# Autodesk Inventor assembly: GE-12053
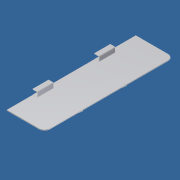
[picture p0: Inventor's stored thumbnail of the model, 180x180]
Saved by Autodesk Inventor 2012 (Build 160160000, 160)
## iProperties
Created: 2011-08-29
Part Number: GE-12053
Document SubType Name: Assembly
Designer: mcyr
Description: Shelf Assembly
Title: Shelf Assembly
Author: mcyr
## Documents named in this file (5)
- C:\Data Folder\FRC 2012 Field\Components\GE-12053.iam
- C:\Data Folder\FRC 2012 Field\Components\GE-12053-02.ipt
- C:\Data Folder\FRC 2012 Field\Components\GE-12053-01.ipt
- C:\Data Folder\FRC 2012 Field\Components\FE-00004-08.iam
- C:\Data Folder\FRC 2012 Field\Components\GE-12052_modified.ipt
## Components (7 placed, 4 different names)
1. GE-12053-02:1 — Mate:1, Flush:1, Mate:2, Flush:2, Flush:3, Mate:4, Flush:4
2. GE-12053-02:2 — Mate:2, Mate:3, Flush:3, Mate:7, Flush:5
3. GE-12053-01:1 — Mate:1, Flush:1, Mate:3, Flush:2, Mate:5, Mate:6, Flush:8, Flush:9, Mate:9, Flush:10, Mate:10, Flush:11
4. FE-00004-08:1 [sub-assembly] — Mate:6, Mate:7, Flush:5
5. FE-00004-08:2 [sub-assembly] — Mate:4, Mate:5, Flush:4
6. GE-12052_modified:1 — Flush:9, Mate:10, Flush:11
7. GE-12052_modified:2 — Flush:8, Mate:9, Flush:10
## Relationships (18: Mate 9, Flush 9)
- Mate:1: GE-12053-02:1 ↔ GE-12053-01:1
- Flush:1 (-400.05 mm): GE-12053-02:1 ↔ GE-12053-01:1
- Mate:2 (406.4 mm): GE-12053-02:1 ↔ GE-12053-02:2
- Mate:3: GE-12053-02:2 ↔ GE-12053-01:1
- Flush:2 (44.45 mm): GE-12053-02:1 ↔ GE-12053-01:1
- Flush:3: GE-12053-02:1 ↔ GE-12053-02:2
- Mate:4: GE-12053-02:1 ↔ FE-00004-08:2
- Mate:5: GE-12053-01:1 ↔ FE-00004-08:2
- Flush:4 (25.4 mm): GE-12053-02:1 ↔ FE-00004-08:2
- Mate:6: GE-12053-01:1 ↔ FE-00004-08:1
- Mate:7: GE-12053-02:2 ↔ FE-00004-08:1
- Flush:5 (25.4 mm): GE-12053-02:2 ↔ FE-00004-08:1
- Flush:8 (241.3 mm): GE-12053-01:1 ↔ GE-12052_modified:2
- Flush:9 (241.3 mm): GE-12053-01:1 ↔ GE-12052_modified:1
- Mate:9: GE-12053-01:1 ↔ GE-12052_modified:2
- Flush:10: GE-12053-01:1 ↔ GE-12052_modified:2
- Mate:10: GE-12053-01:1 ↔ GE-12052_modified:1
- Flush:11: GE-12053-01:1 ↔ GE-12052_modified:1
